# Autodesk Inventor assembly: Worm Gears
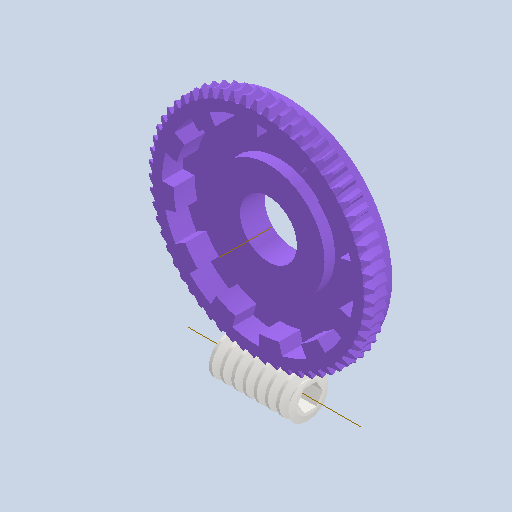
[picture p0: Inventor's stored thumbnail of the model, 512x512]
Saved by Autodesk Inventor 2022 (Build 260153070, 153G)
## iProperties
ClientObjectVersion: 1
Created: 2020-11-06
Part Number: Worm Gears
Document SubType Name: Assembly
Designer: robst
Categories: <?xml version="1.0" encoding="UTF-16"?> <MemberInstance><Categories><FamilyTemplate/><ParamToTemplateMap><ParamToTemplate><ParamToTemplate CategoryParameter="//CategoryParameter[@InternalName='9E91F9C2-1A37-4abf-91CE-B4CF7EE75BC6']" ConstantValue="1000000.000000"/></ParamToTemplate><ParamToTemplate><ParamToTemplate CategoryParameter="//CategoryParameter[@InternalName='2AFF4D85-1BD8-4ea8-8D18-96A2CAB0895B']" ConstantValue="640533.339895"/></ParamToTemplate><ParamToTemplate><ParamToTemplate CategoryParameter="//CategoryParameter[@InternalName='E8E51088-10FD-40b5-B945-790B32C7EFBA']" ConstantValue="104.719755"/></ParamToTemplate><ParamToTemplate><ParamToTemplate CategoryParameter="//CategoryParameter[@InternalName='752D88A1-A866-440c-81C2-59259440B19C']" ConstantValue="1.745329"/></ParamToTemplate><ParamToTemplate><ParamToTemplate CategoryParameter="//CategoryParameter[@InternalName='5F43FD89-24D7-49f6-B63B-C3D8E39D8A69']" ConstantValue="9549.296586"/></ParamToTemplate><ParamToTemplate><ParamToTemplate CategoryParameter="//CategoryParameter[@InternalName='8D239626-6A17-497c-A9EF-C1C80B41D68F']" ConstantValue="366998.570134"/></ParamToTemplate><ParamToTemplate><ParamToTemplate CategoryParameter="//CategoryParameter[@InternalName='41D48E04-51D6-4192-AEE3-C42B8672B6EA']" ConstantValue="0.640533"/></ParamToTemplate><ParamToTemplate><ParamToTemplate CategoryParameter="//CategoryParameter[@InternalName='1E8174DF-B5EE-4822-A5FB-BCD9891126C3']" ConstantValue="10.000000"/></ParamToTemplate><ParamToTemplate><ParamToTemplate CategoryParameter="//CategoryParameter[@InternalName='20F5447C-47B1-4fb0-ACD5-EE92291F3ED6']" ConstantValue="0.505479"/></ParamToTemplate></ParamToTemplateMap><Category DisplayName="Gears" InternalName="3565AA18-AB10-415a-941E-C703DB507537" Mnemonic="Gears"><CategoryParameter DisplayName="P" InternalName="9E91F9C2-1A37-4abf-91CE-B4CF7EE75BC6" Mnemonic="P1"/><CategoryParameter DisplayName="P" InternalName="2AFF4D85-1BD8-4ea8-8D18-96A2CAB0895B" Mnemonic="P2"/><CategoryParameter DisplayName="n" InternalName="E8E51088-10FD-40b5-B945-790B32C7EFBA" Mnemonic="n1"/><CategoryParameter DisplayName="n" InternalName="752D88A1-A866-440c-81C2-59259440B19C" Mnemonic="n2"/><CategoryParameter DisplayName="T" InternalName="5F43FD89-24D7-49f6-B63B-C3D8E39D8A69" Mnemonic="Mk1"/><CategoryParameter DisplayName="T" InternalName="8D239626-6A17-497c-A9EF-C1C80B41D68F" Mnemonic="Mk2"/><CategoryParameter DisplayName="||h|" InternalName="41D48E04-51D6-4192-AEE3-C42B8672B6EA" Mnemonic="eta"/><Category DisplayName="WormGears" InternalName="2B10D032-4568-4ca1-81B6-0EE8891F8531" Mnemonic="WormGears"><CategoryParameter DisplayName="q" InternalName="1E8174DF-B5EE-4822-A5FB-BCD9891126C3" Mnemonic="q"/><CategoryParameter DisplayName="p|.n|" InternalName="20F5447C-47B1-4fb0-ACD5-EE92291F3ED6" Mnemonic="pn"/></Category></Category></Categories></MemberInstance>
Mass: 517.485 g
Surface Area: 307.092 cm^2
Volume: 65.9217 cm^3
Density: 7.85 g/cm^3
Author: robst
## Documents named in this file (3)
- C:\git\CAD-Development\robSteele\ShapeWays\TelescopeProjects\TelescopeMount\forkMountForDecTripV01\Design Accelerator\Worm Gears5.iam
- C:\git\CAD-Development\robSteele\ShapeWays\TelescopeProjects\TelescopeMount\forkMountForDecTripV01\Design Accelerator\Worm5.ipt
- C:\git\CAD-Development\robSteele\ShapeWays\TelescopeProjects\TelescopeMount\forkMountForDecTripV01\Design Accelerator\Worm Gear5.ipt
## Components (2 placed, 2 different names)
1. Worm:1 — Mate:3, Rotation:1
2. Worm Gear:1 — Mate:3, Rotation:1
## Relationships (3: Composite 1, Mate 1, RelateRotation 1)
- [Composite]: Worm:1 ↔ Worm Gear:1
- Mate:3 (56.5955 mm): Worm:1 ↔ Worm Gear:1
- Rotation:1 [RelateRotation] (0.0167 ul): Worm:1 ↔ Worm Gear:1
